# Autodesk Inventor assembly: fin_assembly
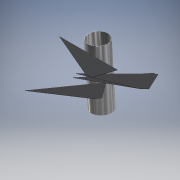
[picture p0: Inventor's stored thumbnail of the model, 180x180]
Saved by Autodesk Inventor 2017 SP1 (Build 210196100, 196)
## iProperties
Created: 2016-10-22
Part Number: fin_assembly
Document SubType Name: Assembly
Designer: cflannery
Author: cflannery
## Documents named in this file (3)
- D:\Triton_Rocket_Club\NONGIT\Vehicles\Intrepid\Structures\fin_assembly.iam
- D:\Triton_Rocket_Club\NONGIT\Vehicles\Intrepid\Structures\fin_can.ipt
- D:\Triton_Rocket_Club\NONGIT\Vehicles\Intrepid\Structures\fin.ipt
## Components (5 placed, 2 different names)
1. fin_can:1 — Tangent:1, Tangent:2, Tangent:3, Tangent:4
2. fin:1 — Tangent:2
3. fin:2 — Tangent:4
4. fin:3 — Tangent:3
5. fin:4 — Tangent:1
## Relationships (4: Tangent 4)
- Tangent:1: fin_can:1 ↔ fin:4
- Tangent:2: fin_can:1 ↔ fin:1
- Tangent:3: fin_can:1 ↔ fin:3
- Tangent:4: fin_can:1 ↔ fin:2
